# Autodesk Inventor assembly: tub_assembled
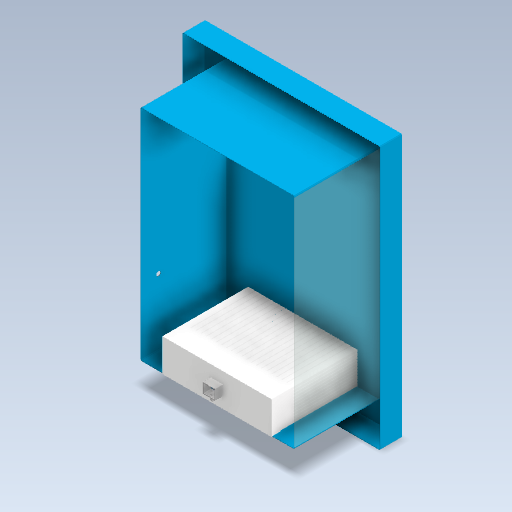
[picture p0: Inventor's stored thumbnail of the model, 512x512]
Saved by Autodesk Inventor 2020 (Build 240168000, 168)
## iProperties
Created: 2020-04-13
Part Number: tub_assembled
Document SubType Name: Assembly
Designer: LENOVO
Author: LENOVO
## Documents named in this file (6)
- C:\Users\LENOVO\Desktop\Graduation Project\Fish Farming Unit\Tub\tub_assembled.iam
- C:\Users\LENOVO\Desktop\Graduation Project\Fish Farming Unit\Tub\tub.ipt
- C:\Users\LENOVO\Desktop\Graduation Project\Fish Farming Unit\Tub\glass_slab.ipt
- C:\Users\LENOVO\Desktop\Graduation Project\Fish Farming Unit\Tub Sensors Holder\Sensors Holder V3.ipt
- C:\Users\LENOVO\Desktop\Graduation Project\Fish Farming Unit\Feeding Mechanism\HC-SR04_ultrasonic.iam
- C:\Users\LENOVO\Desktop\Graduation Project\Fish Farming Unit\Gland\pg7.ipt
## Components (5 placed, 5 different names)
1. tub:2 — Mate:1, Mate:2, Mate:3, Mate:4
2. glass_slab:1 — Mate:1, Mate:2
3. Sensors Holder V3:1 — Mate:3, Mate:4, Insert:1, Insert:2
4. HC-SR04_ultrasonic:1 [sub-assembly] — Insert:1
5. pg7:1 — Insert:2
## Relationships (6: Mate 4, Insert 2)
- Mate:1: tub:2 ↔ glass_slab:1
- Mate:2: tub:2 ↔ glass_slab:1
- Mate:3: tub:2 ↔ Sensors Holder V3:1
- Mate:4: tub:2 ↔ Sensors Holder V3:1
- Insert:1 (-5 mm): Sensors Holder V3:1 ↔ HC-SR04_ultrasonic:1
- Insert:2 (-9.5 mm): Sensors Holder V3:1 ↔ pg7:1
